# Autodesk Inventor assembly: Leg Assembly
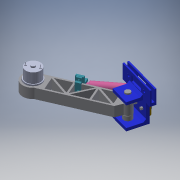
[picture p0: Inventor's stored thumbnail of the model, 180x180]
Saved by Autodesk Inventor 2018 (Build 220112000, 112)
## iProperties
Created: 2018-04-17
Part Number: Leg Assembly
Document SubType Name: Assembly
Designer: MIABo
Author: MIABo
## Documents named in this file (12)
- C:\Users\MIABo\Documents\GitHub\Ares1\3D Model Files\Leg Assembly.iam
- C:\Users\MIABo\Documents\GitHub\Ares1\3D Model Files\Suspension Frame 3.0.ipt
- C:\Users\MIABo\Documents\GitHub\Ares1\3D Model Files\Leg Mount Rivet.ipt
- C:\Users\MIABo\Documents\GitHub\Ares1\3D Model Files\Leg Spacer.ipt
- C:\Users\MIABo\Documents\GitHub\Ares1\3D Model Files\leg 3.0.ipt
- C:\Users\MIABo\Documents\GitHub\Ares1\3D Model Files\SpringPin.ipt
- C:\Users\MIABo\Documents\GitHub\Ares1\3D Model Files\LowerSpringMountRearBracket.ipt
- C:\Users\MIABo\Documents\GitHub\Ares1\3D Model Files\LowerSpringMountFront.ipt
- C:\Users\MIABo\Documents\GitHub\Ares1\3D Model Files\Upper_Spring_Hanger2.ipt
- C:\Users\MIABo\Documents\GitHub\Ares1\3D Model Files\MockShock2.ipt
- C:\Users\MIABo\Documents\GitHub\Ares1\3D Model Files\wheel motor.ipt
- C:\Users\MIABo\Documents\GitHub\Ares1\3D Model Files\Frame mount rivet.ipt
## Components (14 placed, 11 different names)
1. Suspension Frame 3.0:1
2. Leg Mount Rivet:1
3. Leg Spacer:1
4. Leg Spacer:2
5. leg 3.0:1
6. SpringPin:1
7. SpringPin:2
8. LowerSpringMountRearBracket:1
9. LowerSpringMountFront:1
10. Upper_Spring_Hanger2:1
11. MockShock2:1
12. wheel motor:1
13. Frame mount rivet:1
14. Frame mount rivet:2
## Relationships (20: Insert 9, Tangent 6, Mate 5)
- [Insert]: Suspension Frame 3.0:1 ↔ Leg Mount Rivet:1
- [Insert]: Suspension Frame 3.0:1 ↔ Leg Spacer:1
- [Insert]: Leg Spacer:1 ↔ leg 3.0:1
- [Mate]: leg 3.0:1 ↔ LowerSpringMountRearBracket:1
- [Mate]: leg 3.0:1 ↔ LowerSpringMountRearBracket:1
- [Mate]: LowerSpringMountRearBracket:1 ↔ LowerSpringMountFront:1
- [Tangent]: LowerSpringMountRearBracket:1 ↔ LowerSpringMountFront:1
- [Tangent]: LowerSpringMountRearBracket:1 ↔ LowerSpringMountFront:1
- [Insert]: SpringPin:2 ↔ LowerSpringMountFront:1
- [Mate]: Suspension Frame 3.0:1 ↔ Upper_Spring_Hanger2:1
- [Tangent]: Suspension Frame 3.0:1 ↔ Upper_Spring_Hanger2:1
- [Tangent]: Suspension Frame 3.0:1 ↔ Upper_Spring_Hanger2:1
- [Insert]: SpringPin:1 ↔ Upper_Spring_Hanger2:1
- [Insert]: Upper_Spring_Hanger2:1 ↔ MockShock2:1
- [Tangent]: SpringPin:2 ↔ MockShock2:1
- [Mate]: leg 3.0:1 ↔ LowerSpringMountRearBracket:1
- [Insert]: leg 3.0:1 ↔ wheel motor:1
- [Tangent]: leg 3.0:1 ↔ wheel motor:1
- [Insert]: Upper_Spring_Hanger2:1 ↔ Frame mount rivet:2
- [Insert]: Upper_Spring_Hanger2:1 ↔ Frame mount rivet:1
